# Autodesk Inventor assembly: head_right
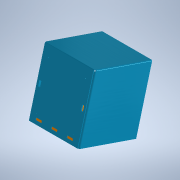
[picture p0: Inventor's stored thumbnail of the model, 180x180]
Saved by Autodesk Inventor 2021.1 (Build 251245010, 245A)
## iProperties
Created: 2023-01-13
Part Number: head_right
Document SubType Name: Assembly
Designer: zmoze
Author: zmoze
## Documents named in this file (3)
- C:\Users\zmoze\OneDrive\Рабочий стол\GrabCAD\Smile_2022-2023\head_right.iam
- C:\Users\zmoze\OneDrive\Рабочий стол\GrabCAD\Smile_2022-2023\face_right.ipt
- C:\Users\zmoze\OneDrive\Рабочий стол\GrabCAD\Smile_2022-2023\head_without_face_right.ipt
## Components (2 placed, 2 different names)
1. face_right:1 — Совмещение:1, Совмещение:2, Совмещение:3, Заподлицо:1
2. head_without_face_right:1 — Совмещение:1, Совмещение:2, Совмещение:3, Заподлицо:1
## Relationships (4: Mate 3, Flush 1)
- Совмещение:1 [Mate]: face_right:1 ↔ head_without_face_right:1
- Совмещение:2 [Mate]: face_right:1 ↔ head_without_face_right:1
- Совмещение:3 [Mate]: face_right:1 ↔ head_without_face_right:1
- Заподлицо:1 [Flush]: face_right:1 ↔ head_without_face_right:1
